# Autodesk Inventor assembly: SteelM-StarS-front-right
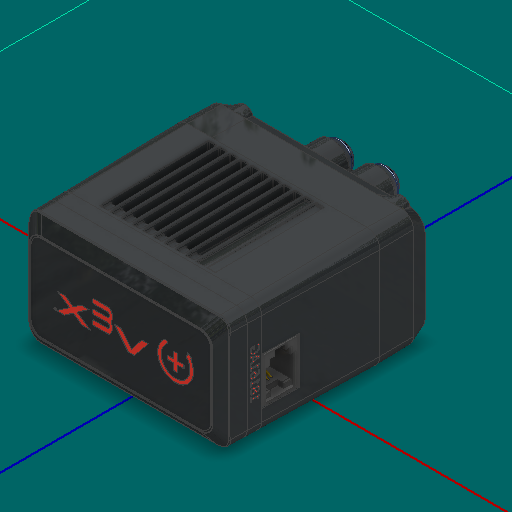
[picture p0: Inventor's stored thumbnail of the model, 512x512]
Saved by Autodesk Inventor 2025 (Build 290162000, 162)
## iProperties
Created: 2022-08-18
Part Number: SteelM-StarS-front-right
Document SubType Name: Assembly
Designer: averey
Author: ylu12
## Documents named in this file (4)
- C:\Users\avere\rbp_cad\atlas\chassis\drive-pod-front-right\SteelM-StarS-front-right.iam
- C:\Users\avere\rbp_cad\atlas\chassis\drive-pod-front-right\V5 Motor-front-right.ipt
- C:\Users\avere\rbp_cad\VEX-CAD-Inventor-1.41\Structure\Hardware\Screw Steel - Star\SScrew Star Smooth .500.ipt
- C:\Users\avere\rbp_cad\VEX-CAD-Inventor-1.41\Structure\Hardware\Screw Steel - Star.ipt
## Components (3 placed, 2 different names)
1. V5 Motor-front-right:1
2. SScrew Star Smooth .500:1
3. SScrew Star Smooth .500:2
## Named parameters: Thickness = 1.1938 mm
